# Autodesk Inventor assembly: Deska Sestava
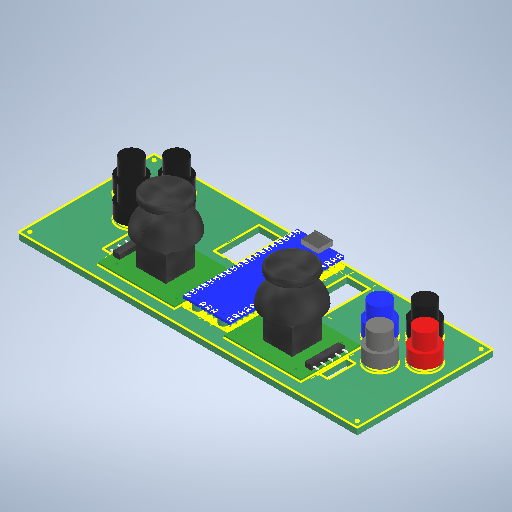
[picture p0: Inventor's stored thumbnail of the model, 512x512]
Saved by Autodesk Inventor 2025 (Build 290162000, 162)
## iProperties
Created: 2024-04-21
Part Number: Deska Sestava
Document SubType Name: Assembly
Designer: domin
Author: domin
## Documents named in this file (5)
- C:\Users\dande\Downloads\Deska_Sestava.iam
- C:\Users\dande\Downloads\stredni_deska.ipt
- C:\Users\dande\Downloads\Joystick.ipt
- C:\Users\dande\Downloads\Raspberry_Pi_Pico.ipt
- C:\Users\dande\Downloads\tlacitko.ipt
## Components (12 placed, 4 different names)
1. stredni_deska:1 — Proti sobě:1, Proti sobě:2, Proti sobě:3, Proti sobě:4, Proti sobě:5, Proti sobě:6, Proti sobě:9, Proti sobě:10, Proti sobě:11, Proti sobě:12, Proti sobě:13, Proti sobě:14, Proti sobě:15, Proti sobě:16, Proti sobě:17, Proti sobě:18, Proti sobě:19, Proti sobě:20, Proti sobě:21, Proti sobě:22, Proti sobě:23, Proti sobě:24, Proti sobě:25, Proti sobě:26, Proti sobě:27, Proti sobě:28, Proti sobě:29, Proti sobě:30, Proti sobě:31, Proti sobě:32, Proti sobě:33, Proti sobě:34, Proti sobě:35
2. Joystick:1 — Proti sobě:1, Proti sobě:2, Proti sobě:6
3. Joystick:2 — Proti sobě:3, Proti sobě:4, Proti sobě:5
4. Raspberry_Pi_Pico:1 — Proti sobě:9, Proti sobě:10, Proti sobě:11
5. tlacitko:1 — Proti sobě:12, Proti sobě:16, Proti sobě:17
6. tlacitko:2 — Proti sobě:13, Proti sobě:18, Proti sobě:19
7. tlacitko:3 — Proti sobě:14, Proti sobě:22, Proti sobě:23
8. tlacitko:4 — Proti sobě:15, Proti sobě:20, Proti sobě:21
9. tlacitko:5 — Proti sobě:24, Proti sobě:30, Proti sobě:31
10. tlacitko:6 — Proti sobě:25, Proti sobě:32, Proti sobě:33
11. tlacitko:7 — Proti sobě:26, Proti sobě:34, Proti sobě:35
12. tlacitko:8 — Proti sobě:27, Proti sobě:28, Proti sobě:29
## Relationships (33: Mate 33)
- Proti sobě:1 [Mate]: stredni_deska:1 ↔ Joystick:1
- Proti sobě:2 [Mate]: stredni_deska:1 ↔ Joystick:1
- Proti sobě:3 [Mate]: stredni_deska:1 ↔ Joystick:2
- Proti sobě:4 [Mate]: stredni_deska:1 ↔ Joystick:2
- Proti sobě:5 [Mate]: stredni_deska:1 ↔ Joystick:2
- Proti sobě:6 [Mate]: stredni_deska:1 ↔ Joystick:1
- Proti sobě:9 [Mate]: stredni_deska:1 ↔ Raspberry_Pi_Pico:1
- Proti sobě:10 [Mate]: stredni_deska:1 ↔ Raspberry_Pi_Pico:1
- Proti sobě:11 [Mate]: stredni_deska:1 ↔ Raspberry_Pi_Pico:1
- Proti sobě:12 [Mate]: stredni_deska:1 ↔ tlacitko:1
- Proti sobě:13 [Mate]: stredni_deska:1 ↔ tlacitko:2
- Proti sobě:14 [Mate]: stredni_deska:1 ↔ tlacitko:3
- Proti sobě:15 [Mate]: stredni_deska:1 ↔ tlacitko:4
- Proti sobě:16 [Mate]: stredni_deska:1 ↔ tlacitko:1
- Proti sobě:17 [Mate]: stredni_deska:1 ↔ tlacitko:1
- Proti sobě:18 [Mate]: stredni_deska:1 ↔ tlacitko:2
- Proti sobě:19 [Mate]: stredni_deska:1 ↔ tlacitko:2
- Proti sobě:20 [Mate]: stredni_deska:1 ↔ tlacitko:4
- Proti sobě:21 [Mate]: stredni_deska:1 ↔ tlacitko:4
- Proti sobě:22 [Mate]: stredni_deska:1 ↔ tlacitko:3
- Proti sobě:23 [Mate]: stredni_deska:1 ↔ tlacitko:3
- Proti sobě:24 [Mate]: stredni_deska:1 ↔ tlacitko:5
- Proti sobě:25 [Mate]: stredni_deska:1 ↔ tlacitko:6
- Proti sobě:26 [Mate]: stredni_deska:1 ↔ tlacitko:7
- Proti sobě:27 [Mate]: stredni_deska:1 ↔ tlacitko:8
- Proti sobě:28 [Mate]: stredni_deska:1 ↔ tlacitko:8
- Proti sobě:29 [Mate]: stredni_deska:1 ↔ tlacitko:8
- Proti sobě:30 [Mate]: stredni_deska:1 ↔ tlacitko:5
- Proti sobě:31 [Mate]: stredni_deska:1 ↔ tlacitko:5
- Proti sobě:32 [Mate]: stredni_deska:1 ↔ tlacitko:6
- Proti sobě:33 [Mate]: stredni_deska:1 ↔ tlacitko:6
- Proti sobě:34 [Mate]: stredni_deska:1 ↔ tlacitko:7
- Proti sobě:35 [Mate]: stredni_deska:1 ↔ tlacitko:7
